# Autodesk Inventor assembly: Raspberry_Pi4 v19
(part 2 of 2)
184. Raspberry Pi 379:1
185. Raspberry Pi 380:1
186. Raspberry Pi 381:1
187. Raspberry Pi 382:1
188. Raspberry Pi 383:1
189. Raspberry Pi 385:1
190. Raspberry Pi 386:1
191. Raspberry Pi 387:1
192. Raspberry Pi 388:1
193. Raspberry Pi 390:1
194. Raspberry Pi 391:1
195. Raspberry Pi 393:1
196. Raspberry Pi 394:1
197. Raspberry Pi 395:1
198. Raspberry Pi 396:1
199. Raspberry Pi 397:1
200. Raspberry Pi 398:1
201. Raspberry Pi 399:1
202. Raspberry Pi 3100:1
203. Raspberry Pi 3101:1
204. Raspberry Pi 3102:1
205. Raspberry Pi 3103:1
206. Raspberry Pi 3104:1
207. Raspberry Pi 3105:1
208. Raspberry Pi 3106:1
209. Raspberry Pi 3107:1
210. Raspberry Pi 3108:1
211. Raspberry Pi 3109:1
212. Raspberry Pi 3110:1
213. Raspberry Pi 3111:1
214. Raspberry Pi 3112:1
215. Raspberry Pi 3113:1
216. Raspberry Pi 3114:1
217. Raspberry Pi 3115:1
218. Raspberry Pi 3116:1
219. Raspberry Pi 3117:1
220. Raspberry Pi 3118:1
221. Raspberry Pi 3119:1
222. Raspberry Pi 3120:1
223. Raspberry Pi 3121:1
224. Raspberry Pi 3122:1
225. Raspberry Pi 3123:1
226. Raspberry Pi 3124:1
227. Raspberry Pi 3125:1
228. Raspberry Pi 3126:1
229. Raspberry Pi 3127:1
230. Raspberry Pi 3128:1
231. Raspberry Pi 3129:1
232. Raspberry Pi 3130:1
233. Raspberry Pi 3131:1
234. Raspberry Pi 3132:1
235. Raspberry Pi 3133:1
236. Raspberry Pi 3134:1
237. Raspberry Pi 3135:1
238. Raspberry Pi 3137:1
239. Raspberry Pi 3138:1
240. Raspberry Pi 3139:1
241. Raspberry Pi 3140:1
242. Raspberry Pi 3141:1
243. Raspberry Pi 3142:1
244. Raspberry Pi 3143:1
245. Raspberry Pi 3144:1
246. Raspberry Pi 3146:1
247. Raspberry Pi 3147:1
248. Raspberry Pi 3149:1
249. Raspberry Pi 3150:1
250. Raspberry Pi 3151:1
251. Raspberry Pi 3152:1
252. Raspberry Pi 3153:1
253. Raspberry Pi 3154:1
254. Raspberry Pi 3155:1
255. Raspberry Pi 3156:1
256. Raspberry Pi 3158:1
257. Raspberry Pi 3159:1
258. Raspberry Pi 3160:1
259. Raspberry Pi 3161:1
260. Raspberry Pi 3162:1
261. Raspberry Pi 3163:1
262. Raspberry Pi 3164:1
263. Raspberry Pi 3165:1
264. Raspberry Pi 3166:1
265. Raspberry Pi 3167:1
266. Raspberry Pi 3168:1
267. Raspberry Pi 3169:1
268. Raspberry Pi 3170:1
269. Raspberry Pi 3171:1
270. Raspberry Pi 3276:1
271. Raspberry Pi 3277:1
272. Raspberry Pi 3278:1
273. Raspberry Pi 3279:1
274. Raspberry Pi 3280:1
275. Raspberry Pi 3281:1
276. Raspberry Pi 3282:1
277. Raspberry Pi 3283:1
278. Raspberry Pi 3284:1
279. Raspberry Pi 3285:1
280. Raspberry Pi 3286:1
281. Raspberry Pi 3287:1
282. Raspberry Pi 3288:1
283. Raspberry Pi 3289:1
284. Raspberry Pi 3290:1
285. Raspberry Pi 3291:1
286. Raspberry Pi 3292:1
287. Raspberry Pi 3293:1
288. Raspberry Pi 3294:1
289. Raspberry Pi 3295:1
290. Raspberry Pi 3296:1
291. Raspberry Pi 3297:1
292. Raspberry Pi 3298:1
293. Raspberry Pi 3299:1
294. Raspberry Pi 3300:1
295. Raspberry Pi 3301:1
296. Raspberry Pi 3302:1
297. Raspberry Pi 3303:1
298. Raspberry Pi 3304:1
299. Raspberry Pi 3305:1
300. Raspberry Pi 3306:1
301. Raspberry Pi 3307:1
302. Raspberry Pi 3308:1
303. Raspberry Pi 3309:1
304. Raspberry Pi 3310:1
305. Raspberry Pi 3311:1
306. Raspberry Pi 3312:1
307. Raspberry Pi 3313:1
308. Raspberry Pi 3314:1
309. Raspberry Pi 3315:1
310. Raspberry Pi 3316:1
311. Raspberry Pi 3317:1
312. Raspberry Pi 3318:1
313. Raspberry Pi 3319:1
314. Raspberry Pi 3320:1
315. Raspberry Pi 3321:1
316. Raspberry Pi 3322:1
317. Raspberry Pi 3323:1
318. Raspberry Pi 3324:1
319. Raspberry Pi 3325:1
320. Raspberry Pi 3326:1
321. Raspberry Pi 3327:1
322. Raspberry Pi 3328:1
323. Raspberry Pi 3329:1
324. Raspberry Pi 3330:1
325. Raspberry Pi 3331:1
326. Raspberry Pi 3332:1
327. Raspberry Pi 3333:1
328. Raspberry Pi 3334:1
329. Raspberry Pi 3335:1
330. Raspberry Pi 3336:1
331. Raspberry Pi 3337:1
332. Raspberry Pi 3338:1
333. Raspberry Pi 3339:1
334. Raspberry Pi 3340:1
335. Raspberry Pi 3341:1
336. Raspberry Pi 3342:1
337. Raspberry Pi 3343:1
338. Raspberry Pi 3344:1
339. Raspberry Pi 3345:1
340. Raspberry Pi 3346:1
341. Raspberry Pi 3347:1
342. Raspberry Pi 3348:1
343. Raspberry Pi 3349:1
344. Raspberry Pi 3350:1
345. Raspberry Pi 3351:1
346. Raspberry Pi 3352:1
347. Raspberry Pi 3353:1
348. Raspberry Pi 3354:1
349. Raspberry Pi 327:2
350. Raspberry Pi 340:2
351. Raspberry Pi 344:2
352. Raspberry Pi 344:3
353. Raspberry Pi 340:3
354. Raspberry Pi 344:4
355. Raspberry Pi 340:4
356. Raspberry Pi 344:5
357. Raspberry Pi 340:5
358. Raspberry Pi 344:6
359. Raspberry Pi 340:6
360. Raspberry Pi 340:7
361. Raspberry Pi 344:7
362. Raspberry Pi 340:8
363. Raspberry Pi 344:8
364. Raspberry Pi 3357:1
365. Raspberry Pi 3355:1
366. Raspberry Pi 3356:1
367. Raspberry Pi 374:2
368. Raspberry Pi 3141:2
369. Raspberry Pi 374:3
370. Raspberry Pi 374:4
371. Raspberry Pi 374:5
372. Part2^Raspberry Pi 3:1
373. Raspberry Pi 3360:1
374. Part4^Raspberry Pi 3:1
375. Raspberry Pi 3159:2
376. Raspberry Pi 3158:2
377. Raspberry Pi 3160:2
378. Raspberry Pi 3162:2
379. Raspberry Pi 3161:2
380. Raspberry Pi 359:2
381. Raspberry Pi 3165:2
382. Raspberry Pi 353:2
383. Raspberry Pi 3164:2
384. Raspberry Pi 3163:2
385. Raspberry Pi 355:2
386. Raspberry Pi 3168:2
387. Raspberry Pi 3170:2
388. Raspberry Pi 3169:2
389. Raspberry Pi 3171:2
390. Raspberry Pi 3167:2
391. Raspberry Pi 3166:2
392. Raspberry Pi 353:3
393. Raspberry Pi 3165:3
394. Raspberry Pi 3163:3
395. Raspberry Pi 3164:3
396. raspberry_pi_B+_(bar_180_2x20):1
397. Solder2:1
398. Solder2_Big:1
399. Solder2_Small:1
400. Solder2_Small:2
401. Solder2_Big:2
402. Solder2_Big:3
403. Solder2_Big:4
404. Solder2_Big:5
405. Solder2_Big:6
406. Solder2_Big:7
407. Solder2_Big:8
408. Raspberry Pi 3359:1
409. Solder2:2
410. Solder2:3
411. Solder2:4
412. Solder2:5
413. Solder2:6
414. Solder2:7
415. Solder2:8
416. Solder2:9
417. Solder2:10
418. Solder2:11
419. Solder2:12
420. Solder2_Big:9
421. mf-msmf050-2:1
422. Solder2_Big:10
423. Raspberry Pi 3163_smaller:1
424. Raspberry Pi 353_smaller:1
425. Raspberry Pi 3164_small:1
426. Raspberry Pi 3165_smaller:1
427. Raspberry Pi 3163_smaller:2
428. Raspberry Pi 353_smaller:2
429. Raspberry Pi 3164_small:2
430. Raspberry Pi 3165_smaller:2
431. Raspberry Pi 3163_smaller:3
432. Raspberry Pi 353_smaller:3
433. Raspberry Pi 3164_small:3
434. Raspberry Pi 3165_smaller:3
435. Raspberry Pi 3141:3
436. Raspberry Pi 3141:4
437. Raspberry Pi 3141:5
438. Raspberry Pi 3141:6
439. Raspberry Pi 3141:7
440. Raspberry Pi 3141:8
441. Raspberry Pi 3141:9
442. Raspberry Pi 3141:10
443. Raspberry Pi 3141:11
444. Raspberry Pi 3141:12
445. Raspberry Pi 3141:13
446. Raspberry Pi 3141:14
447. Raspberry Pi 3141:15
448. Solder2:13
449. Solder2:14
450. Solder2:15
451. Solder2:16
452. Solder2:17
453. Solder2:18
454. Solder2:19
455. Solder2:20
456. Solder2:21
457. Solder2:22
458. Solder2:23
459. Solder2:24
460. Solder2:25
461. Solder2:26
462. Solder2:27
463. Solder2:28
464. Solder2:29
465. Solder2:30
466. Solder2:31
467. Solder2:32
468. Solder2:33
469. Solder2:34
470. Solder2:35
471. Solder2:36
472. Solder2:37
473. Solder2:38
474. Solder2:39
475. Solder2:40
476. Solder2:41
477. Solder2:42
478. Solder2:43
479. Solder2:44
480. Solder2:45
481. Solder2:46
482. Solder2:47
483. Solder2:48
484. Solder2:49
485. Solder2:50
486. Solder2:51
487. Solder2_Small:3
488. Solder2_Small:4
489. Solder2_Small:5
490. Solder2_Small:6
491. Solder2_Small:7
492. Solder2_Small:8
493. Solder2_Small:9
494. Solder2_Small:10
495. Solder2_Small:11
496. Solder2_Small:12
497. Solder2_Small:13
498. Solder2_Small:14
499. Solder2_Small:15
500. Solder2_Small:16
501. Solder2:52
502. Solder2:53
503. Solder2:54
504. Solder2:55
505. Solder2:56
506. Solder2:57
507. Raspberry Pi 3141:16
508. Raspberry Pi 3141:17
509. Raspberry Pi 3141:18
510. Raspberry Pi 3141:19
511. Raspberry Pi 3141:20
512. Raspberry Pi 3141:21
513. Raspberry Pi 3141:22
514. Raspberry Pi 3141:23
515. Raspberry Pi 3141:24
516. Raspberry Pi 3141:25
517. Raspberry Pi 3141:26
518. Raspberry Pi 3141:27
519. Raspberry Pi 3141:28
520. Raspberry Pi 3141:29
521. Raspberry Pi 3141:30
522. Raspberry Pi 3141:31
523. Raspberry Pi 3141:32
524. Raspberry Pi 3141:33
525. Raspberry Pi 3141:34
526. Raspberry Pi 3141:35
527. Raspberry Pi 3141:36
528. Raspberry Pi 3141:37
529. Raspberry Pi 3141:38
530. Raspberry Pi 3141:39
531. Raspberry Pi 3141:40
532. Raspberry Pi 3141:41
533. Raspberry Pi 3141:42
534. Raspberry Pi 3141:43
535. Raspberry Pi 3141:44
536. Raspberry Pi 3141:45
537. Raspberry Pi 3141:46
538. Raspberry Pi 3141:47
539. Raspberry Pi 3141:48
540. Raspberry Pi 3141:49
541. Raspberry Pi 3141:50
542. Raspberry Pi 3141:51
543. Raspberry Pi 3141:52
544. Raspberry Pi 3141:53
545. Raspberry Pi 3141:54
546. Raspberry Pi 3141:55
547. Raspberry Pi 3141:56
548. Raspberry Pi 3141:57
549. Raspberry Pi 3141:58
550. Raspberry Pi 3141:59
551. Raspberry Pi 3141:60
552. Raspberry Pi 374:6
553. Raspberry Pi 3141:61
554. Raspberry Pi 3141:62
555. Raspberry Pi 3141:63
556. Raspberry Pi 3141:64
557. Raspberry Pi 3141:65
558. Raspberry Pi 3141:66
559. Raspberry Pi 3141:67
560. Raspberry Pi 3141:68
561. Raspberry Pi 3141:69
562. Raspberry Pi 3141:70
563. Raspberry Pi 3141:71
564. Raspberry Pi 3141:72
565. Raspberry Pi 3141:73
566. Raspberry Pi 3141:74
567. Raspberry Pi 3141:75
568. Raspberry Pi 3141:76
569. Raspberry Pi 3141:77
570. Raspberry Pi 3141:78
571. Raspberry Pi 3141:79
572. Raspberry Pi 3141:80
573. Raspberry Pi 3141:81
574. Raspberry Pi 3141:82
575. Raspberry Pi 3141:83
576. Raspberry Pi 3141:84
577. Raspberry Pi 3141:85
578. Raspberry Pi 3141:86
579. Raspberry Pi 3141:87
580. Raspberry Pi 3141_smaller:1
581. Raspberry Pi 3141_smaller:2
582. Raspberry Pi 3141_smaller:3
583. Raspberry Pi 3141_smaller:4
584. Raspberry Pi 3141_smaller:5
585. Raspberry Pi 3141_smaller:6
586. Raspberry Pi 3141_smaller:7
587. Raspberry Pi 3141_smaller:8
588. Raspberry Pi 3141_smaller:9
589. Raspberry Pi 3141_smaller:10
590. Raspberry Pi 3141_smaller:11
591. Raspberry Pi 3141_smaller:12
592. Raspberry Pi 3141_smaller:13
593. Raspberry Pi 3141_smaller:14
594. Raspberry Pi 3141_smaller:15
595. Raspberry Pi 3141_smaller:16
596. Raspberry Pi 3141_smaller:17
597. Raspberry Pi 3141_smaller:18
598. Raspberry Pi 3141_smaller:19
599. Raspberry Pi 3141_smaller:20
600. Raspberry Pi 3141_smaller:21
601. Raspberry Pi 3141_smaller:22
602. Raspberry Pi 3141_smaller:23
603. Raspberry Pi 3141_smaller:24
604. Raspberry Pi 3141_smaller:25
605. Raspberry Pi 3281:2
606. Raspberry Pi 3280:2
607. Raspberry Pi 3282:2
608. Raspberry Pi 3285:2
609. Raspberry Pi 3283:2
610. Raspberry Pi 3284:2
611. Raspberry Pi 34:2
612. Raspberry Pi 3141_smaller:26
613. Raspberry Pi 3141_smaller:27
614. Raspberry Pi 3141_smaller:28
615. Raspberry Pi 3141_smaller:29
616. Raspberry Pi 3141_smaller:30
617. Raspberry Pi 3141_smaller:31
618. Raspberry Pi 3141_smaller:32
619. Raspberry Pi 3141_smaller:33
620. Raspberry Pi 3141_smaller:34
621. Raspberry Pi 3141_smaller:35
622. Raspberry Pi 3141_smaller:36
623. Raspberry Pi 3141_smaller:37
624. Raspberry Pi 3141_smaller:38
625. Raspberry Pi 3141_smaller:39
626. Raspberry Pi 3141:88
627. Raspberry Pi 345:2
628. Raspberry Pi 345:3
629. Raspberry Pi 345:4
630. Raspberry Pi 345:5
631. Part1^Raspberry Pi 3:1
632. Raspberry Pi 3141_smaller:40
633. Part1^Raspberry Pi 3:2
634. MOUNT:1
635. 94510A370_Brass Screw-to-Expand Inserts:1
636. 94510A370_Brass Screw-to-Expand Inserts:2
637. 94510A370_Brass Screw-to-Expand Inserts:3
638. 94510A370_Brass Screw-to-Expand Inserts:4
639. 94209A347_Thread-Forming Screws for Soft Metal:1
640. 94209A347_Thread-Forming Screws for Soft Metal:2
641. 94209A347_Thread-Forming Screws for Soft Metal:3
642. 94209A347_Thread-Forming Screws for Soft Metal:4
